# Autodesk Inventor assembly: System_ohne_Grundplatte_links
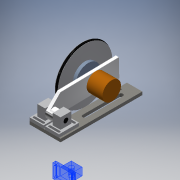
[picture p0: Inventor's stored thumbnail of the model, 180x180]
Saved by Autodesk Inventor 2017 (Build 210142000, 142)
## iProperties
Created: 2017-11-10
Part Number: System_ohne_Grundplatte_links
Document SubType Name: Assembly
Designer: Christoph Soppa
Author: Christoph Soppa
## Documents named in this file (9)
- C:\Users\Nils\Documents\GitHub\Eurobot2018\Hardware\Roboterplatform\Odometrie\System_ohne_Grundplatte_links.iam
- C:\Users\Nils\Documents\GitHub\Eurobot2018\Hardware\Roboterplatform\Odometrie\O Ring 72x3,5x65.ipt
- C:\Users\Nils\Documents\GitHub\Eurobot2018\Hardware\Roboterplatform\Odometrie\Rad d72 b4 r3.5.ipt
- C:\Users\Nils\Documents\GitHub\Eurobot2018\Hardware\Roboterplatform\Odometrie\Drehgeber 2400 .ipt
- C:\Users\Nils\Documents\GitHub\Eurobot2018\Hardware\Roboterplatform\Odometrie\Montageplatte.ipt
- C:\Users\Nils\Documents\GitHub\Eurobot2018\Hardware\Roboterplatform\Odometrie\Stehlager 6mm.ipt
- C:\Users\Nils\Documents\GitHub\Eurobot2018\Hardware\Roboterplatform\Odometrie\6mm Welle.ipt
- C:\Users\Nils\Documents\GitHub\Eurobot2018\Hardware\Roboterplatform\Odometrie\Kupplung.ipt
- C:\Users\Nils\Documents\GitHub\Eurobot2018\Hardware\Roboterplatform\Odometrie\Armlinks.ipt
## Components (9 placed, 8 different names)
1. O Ring 72x3,5x65:1 — Passend:44, Passend:45
2. Rad d72 b4 r3.5:2 — Passend:40, Passend:41, Passend:45
3. Drehgeber 2400 :1 — Passend:36, Passend:37, Passend:38, Passend:39
4. Stehlager 6mm:3 — Passend:30, Passend:33, Passend:34, Passend:35, Fluchtend:11
5. Stehlager 6mm:4 — Passend:29, Fluchtend:9, Fluchtend:10, Passend:31, Passend:32
6. Montageplatte:2 — Passend:29, Passend:30, Fluchtend:9, Fluchtend:10, Fluchtend:12, Passend:46, Passend:47
7. Armlinks:1 — Passend:31, Passend:32, Passend:33, Passend:34, Passend:36, Passend:37
8. Kupplung:2 — Passend:38, Passend:39, Passend:40, Passend:41, Passend:44
9. 6mm Welle:2 — Passend:35, Fluchtend:11
## Relationships (21: Mate 17, Flush 4)
- Passend:29 [Mate]: Stehlager 6mm:4 ↔ Montageplatte:2
- Passend:30 [Mate]: Stehlager 6mm:3 ↔ Montageplatte:2
- Fluchtend:9 [Flush]: Stehlager 6mm:4 ↔ Montageplatte:2
- Fluchtend:10 [Flush]: Stehlager 6mm:4 ↔ Montageplatte:2
- Passend:31 [Mate]: Stehlager 6mm:4 ↔ Armlinks:1
- Passend:32 [Mate]: Stehlager 6mm:4 ↔ Armlinks:1
- Passend:33 [Mate]: Stehlager 6mm:3 ↔ Armlinks:1
- Passend:34 [Mate]: Stehlager 6mm:3 ↔ Armlinks:1
- Passend:35 [Mate]: Stehlager 6mm:3 ↔ 6mm Welle:2
- Fluchtend:11 [Flush]: Stehlager 6mm:3 ↔ 6mm Welle:2
- Passend:36 [Mate]: Drehgeber 2400 :1 ↔ Armlinks:1
- Passend:37 [Mate]: Drehgeber 2400 :1 ↔ Armlinks:1
- Passend:38 [Mate]: Drehgeber 2400 :1 ↔ Kupplung:2
- Passend:39 [Mate]: Drehgeber 2400 :1 ↔ Kupplung:2
- Passend:40 [Mate]: Rad d72 b4 r3.5:2 ↔ Kupplung:2
- Passend:41 [Mate]: Rad d72 b4 r3.5:2 ↔ Kupplung:2
- Passend:44 [Mate]: O Ring 72x3,5x65:1 ↔ Kupplung:2
- Passend:45 [Mate] (-2 mm): O Ring 72x3,5x65:1 ↔ Rad d72 b4 r3.5:2
- Fluchtend:12 [Flush]: Montageplatte:2
- Passend:46 [Mate]: Montageplatte:2
- Passend:47 [Mate]: Montageplatte:2
